# Autodesk Inventor assembly: Assembly1
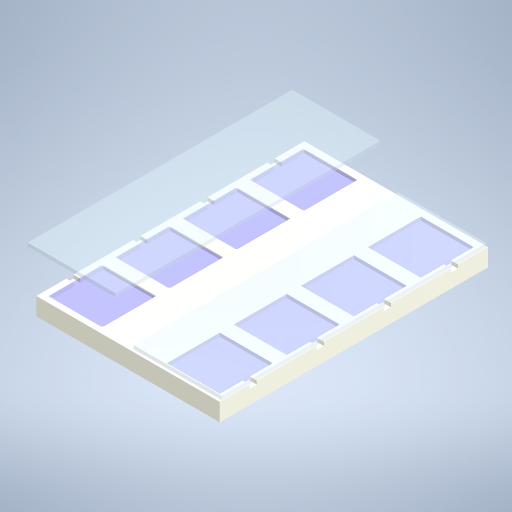
[picture p0: Inventor's stored thumbnail of the model, 512x512]
Saved by Autodesk Inventor 2023 (Build 270158000, 158)
## iProperties
Created: 2023-07-20
Part Number: Assembly1
Document SubType Name: Assembly
Designer: Edwin
Author: Edwin
## Documents named in this file (4)
- E:\Box Sync\Documents\Inventor\Schwartz Laqb\Assembly1.iam
- E:\Box Sync\Documents\Inventor\Schwartz Laqb\slide.ipt
- E:\Box Sync\Documents\Inventor\Schwartz Laqb\GelSlab.ipt
- E:\Box Sync\Documents\Inventor\Schwartz Laqb\MoldForAgaroseOversasd.ipt
## Components (11 placed, 3 different names)
1. slide:1
2. GelSlab:1 — Mate:3, Mate:6
3. GelSlab:2 — Mate:2, Mate:3, Mate:5, Mate:6
4. GelSlab:3 — Mate:1, Mate:2, Mate:4
5. GelSlab:4 — Mate:1, Mate:4, Mate:5
6. MoldForAgaroseOversasd:1
7. GelSlab:5
8. GelSlab:6
9. GelSlab:7
10. GelSlab:8
11. slide:2
## Relationships (12: Mate 12)
- Mate:1: GelSlab:3 ↔ GelSlab:4
- Mate:2: GelSlab:2 ↔ GelSlab:3
- Mate:3: GelSlab:1 ↔ GelSlab:2
- Mate:4 (19.05 mm): GelSlab:3 ↔ GelSlab:4
- Mate:5 (19.05 mm): GelSlab:2 ↔ GelSlab:4
- Mate:6 (19.05 mm): GelSlab:1 ↔ GelSlab:2
- [Mate]: GelSlab:7 ↔ GelSlab:8
- [Mate]: GelSlab:6 ↔ GelSlab:7
- [Mate]: GelSlab:5 ↔ GelSlab:6
- [Mate] (19.05 mm): GelSlab:7 ↔ GelSlab:8
- [Mate] (19.05 mm): GelSlab:6 ↔ GelSlab:8
- [Mate] (19.05 mm): GelSlab:5 ↔ GelSlab:6
## Named parameters: d7_d2 = 0 mm, d8_d4 = 19.05 mm, d9_d5 = 19.05 mm, d10_d6 = 19.05 mm, d11_d0 = 0 mm, d12_d1 = 0 mm
